# Autodesk Inventor assembly: 15102898-16-A-0500
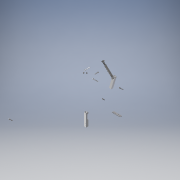
[picture p0: Inventor's stored thumbnail of the model, 180x180]
Saved by Autodesk Inventor 2017 (Build 210142000, 142)
## iProperties
Created: 2016-10-08
Part Number: 15102898-16-A-0500
Document SubType Name: Assembly
Designer: 15102898
Author: 15102898
## Documents named in this file (10)
- C:\Users\15102898\Documents\GitHub\bps-bunnybots2016-cad\Bunnybot-To_be_renamed\15102898-16-A-0000\15102898-16-A-0500.iam
- C:\Users\15102898\Documents\GitHub\bps-bunnybots2016-cad\Bunnybot-To_be_renamed\15102898-16-A-0000\15102898-16-A-0500\15102898-16-A-0501.iam
- C:\Users\15102898\Documents\GitHub\bps-bunnybots2016-cad\Bunnybot-To_be_renamed\15102898-16-A-0000\15102898-16-A-0500\15102898-16-A-0502.iam
- C:\Users\15102898\Documents\GitHub\bps-bunnybots2016-cad\Bunnybot-To_be_renamed\15102898-16-A-0000\15102898-16-A-0500\15102898-16-P-0500.ipt
- C:\Users\15102898\Documents\GitHub\bps-bunnybots2016-cad\Bunnybot-To_be_renamed\15102898-16-A-0000\15102898-16-A-0500\15102898-16-P-0503.ipt
- C:\Users\15102898\Documents\GitHub\bps-bunnybots2016-cad\Bunnybot-To_be_renamed\15102898-16-A-0000\15102898-16-P-0505.ipt
- C:\Users\15102898\Documents\GitHub\bps-bunnybots2016-cad\Bunnybot-To_be_renamed\15102898-16-A-0000\15102898-16-A-0500\15102898-16-P-0505.ipt
- C:\Users\15102898\Documents\GitHub\bps-bunnybots2016-cad\Bunnybot-To_be_renamed\15102898-16-A-0000\15102898-16-A-0500\15102898-16-P-0506.ipt
- C:\Users\15102898\Documents\GitHub\bps-bunnybots2016-cad\Bunnybot-To_be_renamed\15102898-16-A-0000\15102898-16-A-0500\15102898-16-P-0509.ipt
- C:\Users\15102898\Documents\GitHub\bps-bunnybots2016-cad\Bunnybot-To_be_renamed\15102898-16-A-0000\15102898-16-A-0500\15102898-16-P-0510.ipt
## Components (14 placed, 8 different names)
1. 15102898-16-A-0501:1 [sub-assembly] — Cylindrical:1, Mate:1, Mate:3, Mate:4
2. 15102898-16-A-0502:1 [sub-assembly] — Cylindrical:1, Cylindrical:2, Mate:23, Mate:25
3. 15102898-16-P-0500:1 — Mate:2, Mate:3
4. 15102898-16-P-0500:2 — Mate:24, Mate:25
5. 15102898-16-P-0500:3 — Mate:32, Mate:35
6. 15102898-16-P-0500:4 — Mate:33, Mate:34
7. 15102898-16-P-0505:1 — Mate:19, Mate:20, Mate:22, Flush:1, Flush:3, Mate:36, Mate:37, Flush:4, Flush:5
8. 15102898-16-P-0505:3 — Mate:1, Mate:2, Mate:4
9. 15102898-16-P-0503:1 — Mate:19, Mate:20, Cylindrical:2, Mate:21, Mate:24
10. 15102898-16-P-0509:1 — Mate:21, Mate:22, Mate:23
11. 15102898-16-P-0510:1 — Flush:1, Mate:32, Mate:33, Mate:37, Flush:4
12. 15102898-16-P-0510:2 — Flush:3, Mate:28, Mate:29, Mate:30, Mate:31, Mate:36, Flush:5
13. 15102898-16-P-0506:1 — Mate:29, Mate:30, Mate:35
14. 15102898-16-P-0506:2 — Mate:28, Mate:31, Mate:34
## Relationships (27: Mate 21, Flush 4, CylindricalJoint 2)
- Cylindrical:1: 15102898-16-A-0501:1 ↔ 15102898-16-A-0502:1
- Mate:1: 15102898-16-A-0501:1 ↔ 15102898-16-P-0505:3
- Mate:2: 15102898-16-P-0500:1 ↔ 15102898-16-P-0505:3
- Mate:3: 15102898-16-A-0501:1 ↔ 15102898-16-P-0500:1
- Mate:4: 15102898-16-A-0501:1 ↔ 15102898-16-P-0505:3
- Mate:19: 15102898-16-P-0505:1 ↔ 15102898-16-P-0503:1
- Mate:20: 15102898-16-P-0505:1 ↔ 15102898-16-P-0503:1
- Cylindrical:2: 15102898-16-A-0502:1 ↔ 15102898-16-P-0503:1
- Mate:21: 15102898-16-P-0503:1 ↔ 15102898-16-P-0509:1
- Mate:22: 15102898-16-P-0505:1 ↔ 15102898-16-P-0509:1
- Mate:23: 15102898-16-A-0502:1 ↔ 15102898-16-P-0509:1
- Mate:24: 15102898-16-P-0500:2 ↔ 15102898-16-P-0503:1
- Mate:25: 15102898-16-A-0502:1 ↔ 15102898-16-P-0500:2
- Flush:1: 15102898-16-P-0505:1 ↔ 15102898-16-P-0510:1
- Flush:3: 15102898-16-P-0505:1 ↔ 15102898-16-P-0510:2
- Mate:28: 15102898-16-P-0510:2 ↔ 15102898-16-P-0506:2
- Mate:29: 15102898-16-P-0510:2 ↔ 15102898-16-P-0506:1
- Mate:30: 15102898-16-P-0510:2 ↔ 15102898-16-P-0506:1
- Mate:31: 15102898-16-P-0510:2 ↔ 15102898-16-P-0506:2
- Mate:32: 15102898-16-P-0500:3 ↔ 15102898-16-P-0510:1
- Mate:33: 15102898-16-P-0500:4 ↔ 15102898-16-P-0510:1
- Mate:34: 15102898-16-P-0500:4 ↔ 15102898-16-P-0506:2
- Mate:35: 15102898-16-P-0500:3 ↔ 15102898-16-P-0506:1
- Mate:36: 15102898-16-P-0505:1 ↔ 15102898-16-P-0510:2
- Mate:37: 15102898-16-P-0505:1 ↔ 15102898-16-P-0510:1
- Flush:4: 15102898-16-P-0505:1 ↔ 15102898-16-P-0510:1
- Flush:5: 15102898-16-P-0505:1 ↔ 15102898-16-P-0510:2
